# Autodesk Inventor assembly: Inlet and valves
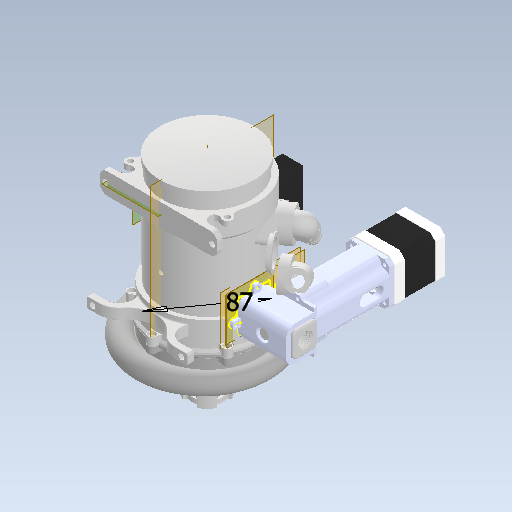
[picture p0: Inventor's stored thumbnail of the model, 512x512]
Saved by Autodesk Inventor 2020 (Build 240168000, 168)
## iProperties
Created: 2020-04-09
Part Number: Inlet and valves
Document SubType Name: Assembly
Designer: angusaitken
Author: angusaitken
## Documents named in this file (14)
- \\Mac\Home\Desktop\3D\Breeze thing\Breeze V2\Inlet subassembly stuff - Angus\Inlet and valves.iam
- \\Mac\Home\Desktop\3D\Breeze thing\Breeze V2\Inlet subassembly stuff - Angus\Inlet housing.ipt
- \\Mac\Home\Desktop\3D\Breeze thing\Breeze V2\Inlet subassembly stuff - Angus\N95 Filter.ipt
- \\Mac\Home\Desktop\3D\Breeze thing\Breeze V2\Inlet subassembly stuff - Angus\HS-322HD servo.ipt
- \\Mac\Home\Desktop\3D\Breeze thing\Breeze V2\Inlet subassembly stuff - Angus\Butterfly valve.ipt
- \\Mac\Home\Desktop\3D\Breeze thing\Breeze V2\Inlet subassembly stuff - Angus\Stepper mount.ipt
- \\Mac\Home\Desktop\3D\Breeze thing\Breeze V2\Inlet subassembly stuff - Angus\4891K720_EASY-SET POLYESTER NEEDLE VALVE.ipt
- \\Mac\Home\Desktop\3D\Breeze thing\Breeze V2\Inlet subassembly stuff - Angus\Valve mount.ipt
- \\Mac\Home\Desktop\3D\Breeze thing\Breeze V2\Inlet subassembly stuff - Angus\NEMA17 stepper motor v40 v1.ipt
- \\Mac\Home\Desktop\3D\Breeze thing\Breeze V2\Inlet subassembly stuff - Angus\Emergency Barb.ipt
- \\Mac\Home\Desktop\3D\Breeze thing\Breeze V2\Impeller Assembly\BRZ-P201.ipt
- \\Mac\Home\Desktop\3D\Breeze thing\Breeze V2\Inlet subassembly stuff - Angus\Emergency barb 45.ipt
- \\Mac\Home\Desktop\3D\Breeze thing\Breeze V2\Impeller Assembly\Impeller Assembly.iam
- \\Mac\Home\Desktop\3D\Breeze thing\Breeze V2\Inlet subassembly stuff - Angus\Inlet 3D print part.iam
## Components (13 placed, 13 different names)
1. Inlet housing:1 — Mate:1, Mate:2, Mate:3, Mate:4, Mate:7, Mate:8, Mate:9, Mate:11, Flush:1, Flush:2, Mate:19, Mate:26, Mate:27, Mate:28, Mate:29, Mate:30, Angle:1, Flush:4, Flush:5, Flush:6
2. N95 Filter:1 — Mate:1, Mate:2
3. HS-322HD servo:1 — Mate:3, Mate:4, Mate:5, Mate:6
4. Butterfly valve:1 — Mate:5, Mate:6
5. Stepper mount:1 — Mate:13, Mate:14, Mate:15, Mate:16, Mate:17, Mate:18
6. 4891K720_EASY-SET POLYESTER NEEDLE VALVE:1 — Mate:11, Mate:12
7. Valve mount:1 — Mate:7, Mate:8, Mate:9, Mate:12, Mate:13, Mate:14, Mate:15, Flush:3
8. NEMA17 stepper motor v40 v1:1 — Mate:16, Mate:17, Mate:18
9. Emergency Barb:1 — Flush:1, Flush:2
10. BRZ-P201:1 — Mate:19
11. Emergency barb 45:2 — Mate:26, Mate:27, Mate:28
12. Impeller Assembly:1 [sub-assembly] — Mate:29, Mate:30, Angle:1, Flush:3, Flush:4, Flush:5, Flush:6, Mate:31, Mate:32, Mate:33
13. Inlet 3D print part:1 [sub-assembly] — Mate:31, Mate:32, Mate:33
## Relationships (33: Mate 26, Flush 6, Angle 1)
- Mate:1: Inlet housing:1 ↔ N95 Filter:1
- Mate:2 (11 mm): Inlet housing:1 ↔ N95 Filter:1
- Mate:3: Inlet housing:1 ↔ HS-322HD servo:1
- Mate:4: Inlet housing:1 ↔ HS-322HD servo:1
- Mate:5: HS-322HD servo:1 ↔ Butterfly valve:1
- Mate:6 (0.5 mm): HS-322HD servo:1 ↔ Butterfly valve:1
- Mate:7: Inlet housing:1 ↔ Valve mount:1
- Mate:8: Inlet housing:1 ↔ Valve mount:1
- Mate:9: Inlet housing:1 ↔ Valve mount:1
- Mate:11: Inlet housing:1 ↔ 4891K720_EASY-SET POLYESTER NEEDLE VALVE:1
- Mate:12: 4891K720_EASY-SET POLYESTER NEEDLE VALVE:1 ↔ Valve mount:1
- Mate:13: Stepper mount:1 ↔ Valve mount:1
- Mate:14: Stepper mount:1 ↔ Valve mount:1
- Mate:15: Stepper mount:1 ↔ Valve mount:1
- Mate:16: Stepper mount:1 ↔ NEMA17 stepper motor v40 v1:1
- Mate:17: Stepper mount:1 ↔ NEMA17 stepper motor v40 v1:1
- Mate:18: Stepper mount:1 ↔ NEMA17 stepper motor v40 v1:1
- Flush:1: Inlet housing:1 ↔ Emergency Barb:1
- Flush:2: Inlet housing:1 ↔ Emergency Barb:1
- Mate:19: Inlet housing:1 ↔ BRZ-P201:1
- Mate:26: Inlet housing:1 ↔ Emergency barb 45:2
- Mate:27: Inlet housing:1 ↔ Emergency barb 45:2
- Mate:28: Inlet housing:1 ↔ Emergency barb 45:2
- Mate:29: Inlet housing:1 ↔ Impeller Assembly:1
- Mate:30: Inlet housing:1 ↔ Impeller Assembly:1
- Angle:1 (0 deg): Inlet housing:1 ↔ Impeller Assembly:1
- Flush:3: Valve mount:1 ↔ Impeller Assembly:1
- Flush:4: Inlet housing:1 ↔ Impeller Assembly:1
- Flush:5: Inlet housing:1 ↔ Impeller Assembly:1
- Flush:6: Inlet housing:1 ↔ Impeller Assembly:1
- Mate:31: Impeller Assembly:1 ↔ Inlet 3D print part:1
- Mate:32: Impeller Assembly:1 ↔ Inlet 3D print part:1
- Mate:33: Impeller Assembly:1 ↔ Inlet 3D print part:1
